# Autodesk Inventor assembly: leg_ass_1_MIR1
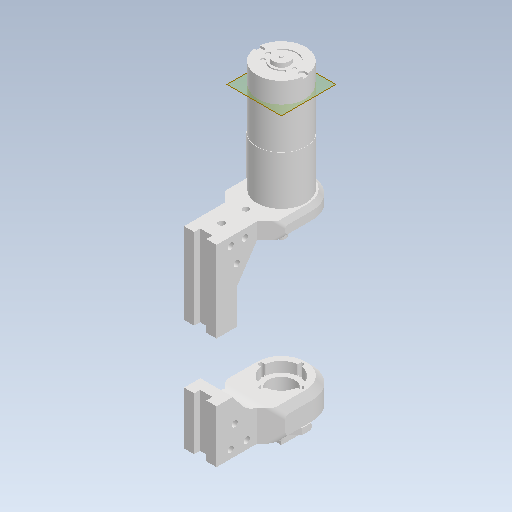
[picture p0: Inventor's stored thumbnail of the model, 512x512]
Saved by Autodesk Inventor 2020 (Build 240168000, 168)
## iProperties
Created: 2019-05-04
Part Number: leg_ass_1_MIR1
Document SubType Name: Assembly
Designer: psrob
Author: psrob
## Documents named in this file (5)
- E:\projects-2\project dog gen2\hardware\leg_ass_1_MIR1.iam
- E:\projects-2\project dog gen2\hardware\dog_bone_1_MIR.ipt
- E:\projects-2\project dog gen2\hardware\motor_2_MIR1.ipt
- E:\projects-2\project dog gen2\hardware\dog_bone_3_MIR.ipt
- E:\projects-2\project dog gen2\hardware\encoder_ass_MIR2.iam
## Components (4 placed, 4 different names)
1. dog_bone_1_MIR:1 — Angle:1, Flush:1, Insert:11, Insert:10
2. motor_2_MIR1:1 — Tangent:1, Mate:1, Flush:2
3. dog_bone_3_MIR:1 — Tangent:1, Angle:1, Mate:1, Flush:1
4. encoder_ass_MIR2:1 [sub-assembly] — Insert:11, Insert:10
## Relationships (7: Flush 2, Insert 2, Tangent 1, Angle 1, Mate 1)
- Tangent:1: motor_2_MIR1:1 ↔ dog_bone_3_MIR:1
- Angle:1 (0 deg): dog_bone_1_MIR:1 ↔ dog_bone_3_MIR:1
- Mate:1: motor_2_MIR1:1 ↔ dog_bone_3_MIR:1
- Flush:1: dog_bone_1_MIR:1 ↔ dog_bone_3_MIR:1
- Insert:11: dog_bone_1_MIR:1 ↔ encoder_ass_MIR2:1
- Insert:10: dog_bone_1_MIR:1 ↔ encoder_ass_MIR2:1
- Flush:2 (-10 mm): motor_2_MIR1:1
